# Autodesk Inventor assembly: Assembly_openSIM_module_v2
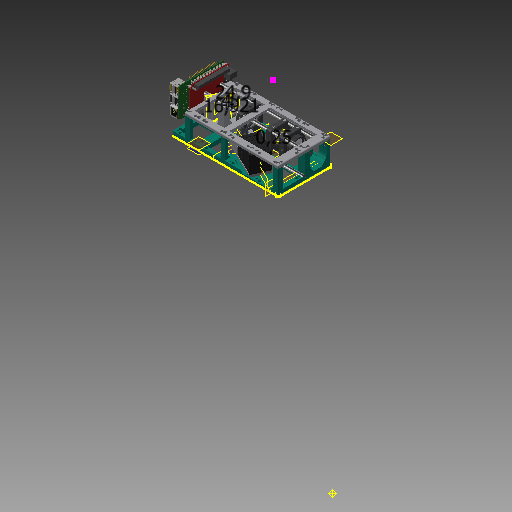
[picture p0: Inventor's stored thumbnail of the model, 512x512]
Saved by Autodesk Inventor 2019 (Build 230136000, 136)
## iProperties
Created: 2019-10-16
Part Number: Assembly_openSIM_module_v2
Document SubType Name: Assembly
Designer: diederichbenedict
Mass: 441.865 g
Surface Area: 2815.17 cm^2
Volume: 441.865 cm^3
Density: 1 g/cm^3
Author: diederichbenedict
## Documents named in this file (17)
- C:\Users\marsikovabarbora\Dropbox\UC2\02_CAD\INVENTOR\uc2_v3\Assembly_openSIM_module.iam
- C:\Users\marsikovabarbora\Dropbox\UC2\02_CAD\INVENTOR\uc2_v3\00_TI_DLP_2000_Chip.ipt
- C:\Users\marsikovabarbora\Dropbox\UC2\02_CAD\INVENTOR\uc2_v3\00_Lens_Iphone_5s.ipt
- C:\Users\marsikovabarbora\Dropbox\UC2\02_CAD\INVENTOR\uc2_v3\00_Thorlabs_Rod_200mm.ipt
- C:\Users\marsikovabarbora\Dropbox\UC2\02_CAD\INVENTOR\uc2_v3\00_CUBE_openSIM_LA1131-ML-Step.ipt
- C:\Users\marsikovabarbora\Dropbox\UC2\02_CAD\INVENTOR\uc2_v3\00_Thorlabs_Cage_CP33_M.ipt
- C:\Users\marsikovabarbora\Dropbox\UC2\02_CAD\INVENTOR\uc2_v3\30_CUBE_openSIM_Laser_Telescope_Mount.ipt
- C:\Users\marsikovabarbora\Dropbox\UC2\02_CAD\INVENTOR\uc2_v3\00_CUBE_openSIM_Beamexpander_Lens_20mm_Edmundoptics.ipt
- C:\Users\marsikovabarbora\Dropbox\UC2\02_CAD\INVENTOR\uc2_v3\30_CUBE_openSIM_Cagelid.ipt
- C:\Users\marsikovabarbora\Dropbox\UC2\02_CAD\INVENTOR\uc2_v3\30_Cube_openSIM_Fouriermask.ipt
- C:\Users\marsikovabarbora\Dropbox\UC2\02_CAD\INVENTOR\uc2_v3\30_CUBE_openSIM_base_v4.ipt
- C:\Users\marsikovabarbora\Dropbox\UC2\02_CAD\INVENTOR\uc2_v3\30_CUBE_openSIM_DMD_Holder.ipt
- C:\Users\marsikovabarbora\Dropbox\UC2\02_CAD\INVENTOR\uc2_v3\30_CUBE_openSIM_Rodholder.ipt
- C:\Users\marsikovabarbora\Dropbox\UC2\02_CAD\INVENTOR\uc2_v3\30_CUBE_openSIM_DMD_Fixation_base.ipt
- C:\Users\marsikovabarbora\Dropbox\UC2\02_CAD\INVENTOR\uc2_v3\00_LASER_640nm.ipt
- C:\Users\marsikovabarbora\Dropbox\UC2\02_CAD\INVENTOR\uc2_v3\00_Raspi.ipt
- C:\Users\marsikovabarbora\Dropbox\UC2\02_CAD\INVENTOR\uc2_v3\00_TI_DLP_2000EVM.ipt
## Components (21 placed, 16 different names)
1. 30_CUBE_openSIM_base_v4:1 — Mate:29, Flush:3, Mate:58, Mate:59, Mate:60, Angle:1, Mate:78, Mate:86, Mate:88, Mate:89, Flush:7, Mate:99, Mate:111, Mate:112, Mate:113, Mate:114, Mate:115, Mate:116
2. 00_TI_DLP_2000_Chip:1 — Mate:105, Mate:106, Mate:108
3. 00_Thorlabs_Rod_200mm:2 — Mate:29, Flush:3
4. 00_CUBE_openSIM_LA1131-ML-Step:1 — Mate:34, Mate:35
5. 00_CUBE_openSIM_LA1131-ML-Step:2 — Mate:32, Mate:33
6. 30_Cube_openSIM_Fouriermask:1 — Mate:79, Flush:8
7. 00_Lens_Iphone_5s:1 — Mate:65, Angle:1, Mate:66, Mate:68
8. 00_CUBE_openSIM_Beamexpander_Lens_20mm_Edmundoptics:1 — Mate:67, Mate:68
9. 00_Thorlabs_Cage_CP33_M:1 — Mate:32, Mate:33, Mate:74, Mate:79, Mate:85, Mate:100
10. 00_Thorlabs_Cage_CP33_M:3 — Mate:34, Mate:35, Mate:78, Mate:85, Mate:104
11. 30_CUBE_openSIM_Laser_Telescope_Mount:1 — Mate:55, Mate:56, Mate:57, Mate:58, Mate:59, Mate:60, Mate:67
12. 00_LASER_640nm:1 — Mate:55, Mate:56, Mate:57, Mate:65, Mate:66
13. 00_Thorlabs_Rod_200mm:3 — Mate:74, Flush:7, Mate:99, Mate:102, Mate:103, Mate:104
14. 30_CUBE_openSIM_Lid:1 — Mate:86, Mate:88, Angle:2
15. 00_Thorlabs_Rod_200mm:4 — Mate:89, Mate:100, Mate:101
16. 00_Thorlabs_Cage_CP33_M:2 — Mate:101, Mate:102, Flush:8, Mate:103
17. 30_openSIM_DMD_Holder:1 — Mate:105, Mate:106, Mate:107, Mate:108, Mate:109, Mate:110
18. 30_openSIM_Rodholder:1 — Mate:114, Mate:115, Mate:116, Flush:9
19. 30_openSIM_DMD_Fixation_base:1 — Mate:107, Mate:109, Mate:110, Mate:111, Mate:112, Mate:113, Mate:117
20. 00_Raspi:1 — Flush:10, Flush:11, Flush:12
21. 00_TI_DLP_2000EVM:1 — Mate:117, Angle:2, Flush:9, Flush:10, Flush:11, Flush:12
## Relationships (50: Mate 41, Flush 7, Angle 2)
- Mate:29: 30_CUBE_openSIM_base_v4:1 ↔ 00_Thorlabs_Rod_200mm:2
- Flush:3: 30_CUBE_openSIM_base_v4:1 ↔ 00_Thorlabs_Rod_200mm:2
- Mate:32: 00_CUBE_openSIM_LA1131-ML-Step:2 ↔ 00_Thorlabs_Cage_CP33_M:1
- Mate:33: 00_CUBE_openSIM_LA1131-ML-Step:2 ↔ 00_Thorlabs_Cage_CP33_M:1
- Mate:34: 00_CUBE_openSIM_LA1131-ML-Step:1 ↔ 00_Thorlabs_Cage_CP33_M:3
- Mate:35: 00_CUBE_openSIM_LA1131-ML-Step:1 ↔ 00_Thorlabs_Cage_CP33_M:3
- Mate:55: 30_CUBE_openSIM_Laser_Telescope_Mount:1 ↔ 00_LASER_640nm:1
- Mate:56: 30_CUBE_openSIM_Laser_Telescope_Mount:1 ↔ 00_LASER_640nm:1
- Mate:57: 30_CUBE_openSIM_Laser_Telescope_Mount:1 ↔ 00_LASER_640nm:1
- Mate:58: 30_CUBE_openSIM_base_v4:1 ↔ 30_CUBE_openSIM_Laser_Telescope_Mount:1
- Mate:59: 30_CUBE_openSIM_base_v4:1 ↔ 30_CUBE_openSIM_Laser_Telescope_Mount:1
- Mate:60: 30_CUBE_openSIM_base_v4:1 ↔ 30_CUBE_openSIM_Laser_Telescope_Mount:1
- Mate:65: 00_Lens_Iphone_5s:1 ↔ 00_LASER_640nm:1
- Angle:1 (0 deg): 30_CUBE_openSIM_base_v4:1 ↔ 00_Lens_Iphone_5s:1
- Mate:66: 00_Lens_Iphone_5s:1 ↔ 00_LASER_640nm:1
- Mate:67: 00_CUBE_openSIM_Beamexpander_Lens_20mm_Edmundoptics:1 ↔ 30_CUBE_openSIM_Laser_Telescope_Mount:1
- Mate:68 (22 mm): 00_Lens_Iphone_5s:1 ↔ 00_CUBE_openSIM_Beamexpander_Lens_20mm_Edmundoptics:1
- Mate:74: 00_Thorlabs_Cage_CP33_M:1 ↔ 00_Thorlabs_Rod_200mm:3
- Mate:78 (30 mm): 30_CUBE_openSIM_base_v4:1 ↔ 00_Thorlabs_Cage_CP33_M:3
- Mate:79: 30_Cube_openSIM_Fouriermask:1 ↔ 00_Thorlabs_Cage_CP33_M:1
- Mate:85 (70 mm): 00_Thorlabs_Cage_CP33_M:1 ↔ 00_Thorlabs_Cage_CP33_M:3
- Mate:86: 30_CUBE_openSIM_base_v4:1 ↔ 30_CUBE_openSIM_Lid:1
- Mate:88: 30_CUBE_openSIM_base_v4:1 ↔ 30_CUBE_openSIM_Lid:1
- Mate:89: 30_CUBE_openSIM_base_v4:1 ↔ 00_Thorlabs_Rod_200mm:4
- Flush:7 (-22.3 mm): 30_CUBE_openSIM_base_v4:1 ↔ 00_Thorlabs_Rod_200mm:3
- Mate:99: 30_CUBE_openSIM_base_v4:1 ↔ 00_Thorlabs_Rod_200mm:3
- Mate:100: 00_Thorlabs_Cage_CP33_M:1 ↔ 00_Thorlabs_Rod_200mm:4
- Mate:101: 00_Thorlabs_Rod_200mm:4 ↔ 00_Thorlabs_Cage_CP33_M:2
- Mate:102: 00_Thorlabs_Rod_200mm:3 ↔ 00_Thorlabs_Cage_CP33_M:2
- Flush:8 (8 mm): 30_Cube_openSIM_Fouriermask:1 ↔ 00_Thorlabs_Cage_CP33_M:2
- Mate:103: 00_Thorlabs_Rod_200mm:3 ↔ 00_Thorlabs_Cage_CP33_M:2
- Mate:104: 00_Thorlabs_Cage_CP33_M:3 ↔ 00_Thorlabs_Rod_200mm:3
- Mate:105: 00_TI_DLP_2000_Chip:1 ↔ 30_openSIM_DMD_Holder:1
- Mate:106: 00_TI_DLP_2000_Chip:1 ↔ 30_openSIM_DMD_Holder:1
- Mate:107: 30_openSIM_DMD_Holder:1 ↔ 30_openSIM_DMD_Fixation_base:1
- Mate:108: 00_TI_DLP_2000_Chip:1 ↔ 30_openSIM_DMD_Holder:1
- Mate:109 (3 mm): 30_openSIM_DMD_Holder:1 ↔ 30_openSIM_DMD_Fixation_base:1
- Mate:110: 30_openSIM_DMD_Holder:1 ↔ 30_openSIM_DMD_Fixation_base:1
- Mate:111: 30_CUBE_openSIM_base_v4:1 ↔ 30_openSIM_DMD_Fixation_base:1
- Mate:112: 30_CUBE_openSIM_base_v4:1 ↔ 30_openSIM_DMD_Fixation_base:1
- Mate:113: 30_CUBE_openSIM_base_v4:1 ↔ 30_openSIM_DMD_Fixation_base:1
- Mate:114: 30_CUBE_openSIM_base_v4:1 ↔ 30_openSIM_Rodholder:1
- Mate:115: 30_CUBE_openSIM_base_v4:1 ↔ 30_openSIM_Rodholder:1
- Mate:116: 30_CUBE_openSIM_base_v4:1 ↔ 30_openSIM_Rodholder:1
- Mate:117 (8 mm): 30_openSIM_DMD_Fixation_base:1 ↔ 00_TI_DLP_2000EVM:1
- Angle:2 (0 deg): 30_CUBE_openSIM_Lid:1 ↔ 00_TI_DLP_2000EVM:1
- Flush:9: 30_openSIM_Rodholder:1 ↔ 00_TI_DLP_2000EVM:1
- Flush:10 (-25 mm): 00_Raspi:1 ↔ 00_TI_DLP_2000EVM:1
- Flush:11: 00_Raspi:1 ↔ 00_TI_DLP_2000EVM:1
- Flush:12: 00_Raspi:1 ↔ 00_TI_DLP_2000EVM:1
